# Autodesk Inventor assembly: Assembly1
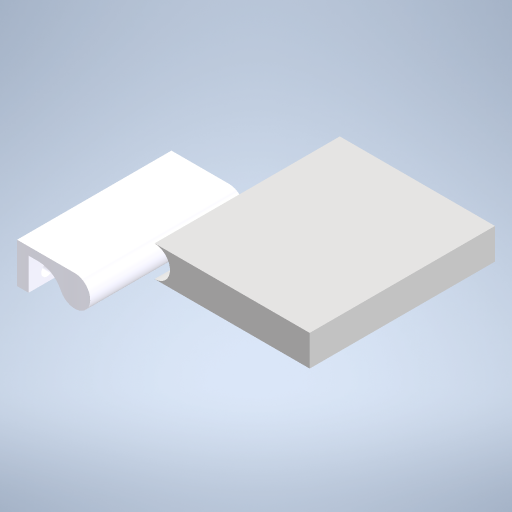
[picture p0: Inventor's stored thumbnail of the model, 512x512]
Saved by Autodesk Inventor 2024.2 (Build 282272000, 272)
## iProperties
Created: 2024-11-21
Part Number: Assembly1
Document SubType Name: Assembly
Designer: Tom
Author: Tom
## Documents named in this file (3)
- C:\Users\Tom\Desktop\UCSF\Preeya UCB\stretchable project\Strain-Sensor-\CAD Files\auto bender part files\Assembly1.iam
- C:\Users\Tom\Desktop\UCSF\Preeya UCB\stretchable project\Strain-Sensor-\CAD Files\auto bender part files\knuckle plate original.ipt
- C:\Users\Tom\Desktop\UCSF\Preeya UCB\stretchable project\Strain-Sensor-\CAD Files\auto bender part files\knuckle plate original mate.ipt
## Components (2 placed, 2 different names)
1. knuckle plate original:1 — Angle:1
2. knuckle plate original mate:1 — Angle:1
## Relationships (1: Angle 1)
- Angle:1 (0 deg): knuckle plate original:1 ↔ knuckle plate original mate:1
